# Autodesk Inventor assembly: baseCarrito2
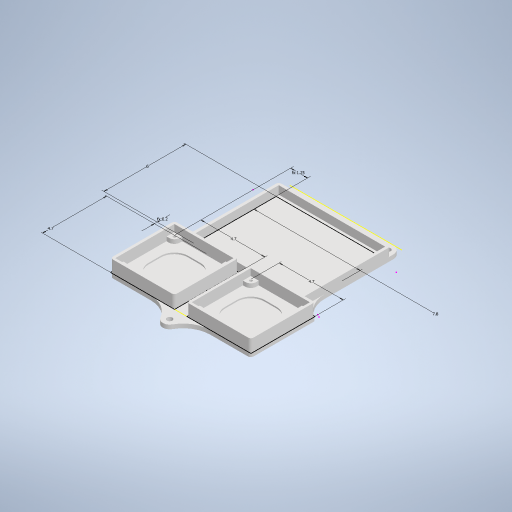
[picture p0: Inventor's stored thumbnail of the model, 512x512]
Saved by Autodesk Inventor 2024 (Build 280153000, 153)
## iProperties
Created: 2024-04-23
Part Number: baseCarrito2
Document SubType Name: Assembly
Designer: Ruki
Author: Ruki
## Documents named in this file (3)
- C:\Users\Public\Documents\Autodesk\Inventor 2024\baseCarrito2.iam
- C:\Users\Ruki\Documents\Inventor\baseCarrito2.ipt
- C:\Users\Ruki\Downloads\bracket.ipt
## Components (3 placed, 2 different names)
1. baseCarrito2:1 — Mate:1, Mate:2, Mate:3, Mate:4
2. bracket:1 — Mate:1, Mate:2
3. bracket:2 — Mate:3, Mate:4
## Relationships (4: Mate 4)
- Mate:1: baseCarrito2:1 ↔ bracket:1
- Mate:2: baseCarrito2:1 ↔ bracket:1
- Mate:3: baseCarrito2:1 ↔ bracket:2
- Mate:4: baseCarrito2:1 ↔ bracket:2
